# Autodesk Inventor assembly: keyboard
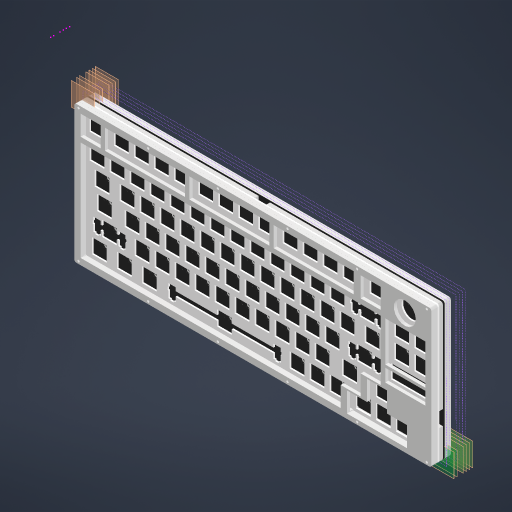
[picture p0: Inventor's stored thumbnail of the model, 512x512]
Saved by Autodesk Inventor 2024.2 (Build 282272000, 272)
## iProperties
Created: 2024-06-20
Part Number: keyboard
Document SubType Name: Assembly
Designer: Moe
Author: Moe
## Documents named in this file (12)
- D:\Code\git\Model-B\case\models\keyboard.iam
- D:\Code\git\Model-B\case\models\swplate.ipt
- D:\Code\git\Model-B\case\models\top-layer.ipt
- D:\Code\git\Model-B\case\models\open_liner.ipt
- D:\Code\git\Model-B\case\models\model-b-pcb.ipt
- D:\Code\git\Model-B\case\models\closed_liner.ipt
- D:\Code\git\Model-B\case\models\rear_plate.ipt
- D:\Code\git\Model-B\case\models\foot1.ipt
- D:\Code\git\Model-B\case\models\foot2.ipt
- D:\Code\git\Model-B\case\models\foot3.ipt
- D:\Code\git\Model-B\case\models\foot4.ipt
- D:\Code\git\Model-B\case\models\top_plate.ipt
## Components (11 placed, 11 different names)
1. swplate:1 — Mate:1, Mate:2, Mate:12, Mate:13
2. top-layer:1 — Mate:1, Mate:11, Mate:13
3. open_liner:1 — Mate:2, Mate:12, Mate:14
4. closed_liner:1 — Mate:5, Mate:15
5. rear_plate:1 — Mate:5, Mate:7
6. foot1:1 — Mate:7, Mate:8
7. foot2:1 — Mate:8, Mate:9
8. foot3:1 — Mate:9, Mate:10
9. foot4:1 — Mate:10
10. top_plate:1 — Mate:11
11. model-b-pcb:1 — Mate:14, Mate:15
## Relationships (12: Mate 12)
- Mate:1: swplate:1 ↔ top-layer:1
- Mate:2: swplate:1 ↔ open_liner:1
- Mate:5: closed_liner:1 ↔ rear_plate:1
- Mate:7: rear_plate:1 ↔ foot1:1
- Mate:8: foot1:1 ↔ foot2:1
- Mate:9: foot2:1 ↔ foot3:1
- Mate:10: foot3:1 ↔ foot4:1
- Mate:11: top-layer:1 ↔ top_plate:1
- Mate:12: swplate:1 ↔ open_liner:1
- Mate:13: swplate:1 ↔ top-layer:1
- Mate:14: open_liner:1 ↔ model-b-pcb:1
- Mate:15: closed_liner:1 ↔ model-b-pcb:1
## Named parameters: Finish10_Area = 1217.94, Finish16_Area = 640.413, Finish1_Area = 45.1814, Finish2_Area = 7.38, Finish3_Area = 24.4601, Finish4_Area = 68.6655, Finish5_Area = 0.0942477, Finish6_Area = 66.4549, Finish7_Area = 889.514, Finish8_Area = 1168.75, Finish9_Area = 55.6977
note: some values were not read from the file. Shown as the stored number, unit unknown: "Finish10_Area", "Finish16_Area", "Finish1_Area", "Finish2_Area", "Finish3_Area", "Finish4_Area", "Finish5_Area", "Finish6_Area", "Finish7_Area", "Finish8_Area", "Finish9_Area".
